# Autodesk Inventor assembly: Assembly3
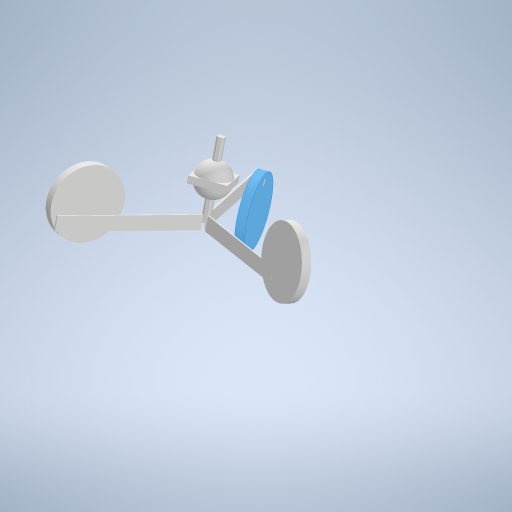
[picture p0: Inventor's stored thumbnail of the model, 512x512]
Saved by Autodesk Inventor 2024 (Build 280153000, 153)
## iProperties
Created: 2024-01-15
Part Number: Assembly3
Document SubType Name: Assembly
Designer: Owner
Author: Owner
## Documents named in this file (5)
- C:\Users\Owner\PycharmProjects\DodgeBot\CAD_FILES\Assembly3.iam
- C:\Users\Owner\PycharmProjects\DodgeBot\CAD_FILES\Ball Joint.ipt
- C:\Users\Owner\PycharmProjects\DodgeBot\CAD_FILES\Post.ipt
- C:\Users\Owner\PycharmProjects\DodgeBot\CAD_FILES\Wheel_Consept.ipt
- C:\Users\Owner\PycharmProjects\DodgeBot\CAD_FILES\Belt.ipt
## Components (9 placed, 4 different names)
1. Ball Joint:1 — Ball:1
2. Post:1 — Rigid:1, Rigid:2, Rigid:3, Rigid:4
3. Post:2 — Ball:1, Rigid:1
4. Wheel_Consept:1 — Rotational:1
5. Belt:2 — Rotational:1, Rigid:3
6. Wheel_Consept:2
7. Belt:3 — Rigid:4
8. Wheel_Consept:3
9. Belt:4 — Rigid:2
## Relationships (8: WeldJoint 4, RevoluteJoint 3, BallJoint 1)
- Ball:1: Ball Joint:1 ↔ Post:2
- Rigid:1 [WeldJoint]: Post:1 ↔ Post:2
- Rotational:1 [RevoluteJoint]: Wheel_Consept:1 ↔ Belt:2
- [RevoluteJoint]: Wheel_Consept:2 ↔ Belt:3
- [RevoluteJoint]: Wheel_Consept:3 ↔ Belt:4
- Rigid:2 [WeldJoint]: Post:1 ↔ Belt:4
- Rigid:3 [WeldJoint]: Post:1 ↔ Belt:2
- Rigid:4 [WeldJoint]: Post:1 ↔ Belt:3
## Named parameters: d5_d3 = 0 mm, d6_d4 = -0.150877 deg, d7_d3 = 0 mm, d8_d4 = -149.000999 deg
